# Autodesk Inventor assembly: Lathe Model V3
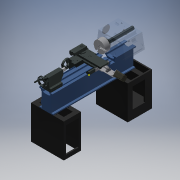
[picture p0: Inventor's stored thumbnail of the model, 180x180]
Saved by Autodesk Inventor 2018 (Build 220112000, 112)
## iProperties
Created: 2017-05-02
Part Number: Lathe Model V3
Document SubType Name: Assembly
Designer: M228544
Author: M228544
## Documents named in this file (28)
- C:\Users\M228299\Documents\GitHub\CNC-Lathe-CAD\CNC Lathe Project\Project Files\Lathe Model 2018.iam
- C:\Users\M228299\Documents\GitHub\CNC-Lathe-CAD\CNC Lathe Project\Project Files\BED.ipt
- C:\Users\M228299\Documents\GitHub\CNC-Lathe-CAD\CNC Lathe Project\Project Files\Bottom-Tool-Bit.ipt
- C:\Users\M228299\Documents\GitHub\CNC-Lathe-CAD\CNC Lathe Project\Project Files\Top-Part-Tool-bit.ipt
- C:\Users\M228299\Documents\GitHub\CNC-Lathe-CAD\CNC Lathe Project\Project Files\tail stock - body part.ipt
- C:\Users\M228299\Documents\GitHub\CNC-Lathe-CAD\CNC Lathe Project\Project Files\Left leg.ipt
- C:\Users\M228299\Documents\GitHub\CNC-Lathe-CAD\CNC Lathe Project\Project Files\Right Leg.ipt
- C:\Users\M228299\Documents\GitHub\CNC-Lathe-CAD\CNC Lathe Project\Project Files\Apron.ipt
- C:\Users\M228299\Documents\GitHub\CNC-Lathe-CAD\CNC Lathe Project\Project Files\Servo Motor\Servo Motor.iam
- C:\Users\M228299\Documents\GitHub\CNC-Lathe-CAD\CNC Lathe Project\Project Files\Ball screw nut and apron join.ipt
- C:\Users\M228299\Documents\GitHub\CNC-Lathe-CAD\CNC Lathe Project\Project Files\barrel.ipt
- C:\Users\M228299\Documents\GitHub\CNC-Lathe-CAD\CNC Lathe Project\Project Files\connecting wheel.ipt
- C:\Users\M228299\Documents\GitHub\CNC-Lathe-CAD\CNC Lathe Project\Project Files\chuck holder.ipt
- C:\Users\M228299\Documents\GitHub\CNC-Lathe-CAD\CNC Lathe Project\Project Files\Chuck shaft.ipt
- C:\Users\M228299\Documents\GitHub\CNC-Lathe-CAD\CNC Lathe Project\Project Files\X axis screw support.ipt
- C:\Users\M228299\Documents\GitHub\CNC-Lathe-CAD\CNC Lathe Project\Project Files\Assembly3.iam
- C:\Users\M228299\Documents\GitHub\CNC-Lathe-CAD\CNC Lathe Project\Project Files\Gearbox Handle.iam
- C:\Users\M228299\Documents\GitHub\CNC-Lathe-CAD\CNC Lathe Project\Project Files\Encoder Mount Hole Plug.ipt
- C:\Users\M228299\Documents\GitHub\CNC-Lathe-CAD\CNC Lathe Project\Project Files\Gearbox.ipt
- C:\Users\M228299\Documents\GitHub\CNC-Lathe-CAD\CNC Lathe Project\Project Files\Encoder Subassembly\Mounting.iam
- C:\Users\M228299\Documents\GitHub\CNC-Lathe-CAD\CNC Lathe Project\Project Files\X-axis Changes\slide-ontop-of-saddle.ipt
- C:\Users\M228299\Documents\GitHub\CNC-Lathe-CAD\CNC Lathe Project\Project Files\X-axis Changes\X Axis Shaft Assembly\short shaft x axis\shaft and nut.iam
- C:\Users\M228299\Documents\GitHub\CNC-Lathe-CAD\CNC Lathe Project\Project Files\X-axis Changes\Ball Screw\Correct nut unmodified ASSembly.iam
- C:\Users\M228299\Documents\GitHub\CNC-Lathe-CAD\CNC Lathe Project\Project Files\X-axis Changes\Ball Screw\X-axis Ball Screw Support.ipt
- C:\Users\M228299\Documents\GitHub\CNC-Lathe-CAD\CNC Lathe Project\Project Files\saddle.ipt
- C:\Users\M228299\Documents\GitHub\CNC-Lathe-CAD\CNC Lathe Project\Project Files\back plate.ipt
- C:\Users\M228299\Documents\GitHub\CNC-Lathe-CAD\CNC Lathe Project\Project Files\front.ipt
- C:\Users\M228299\Documents\GitHub\CNC-Lathe-CAD\CNC Lathe Project\Project Files\polycarbonate cover.ipt
## Components (27 placed, 27 different names)
1. BED:1 — Mate:1, Mate:2, Mate:9, Mate:10, Mate:11, Flush:5, Flush:6, Mate:13, Mate:14, Flush:7, Flush:9
2. saddle:1 — Mate:1, Mate:2, Mate:5, Mate:6, Saddle and Slice on top of saddle, Flush:10, Flush:11, Mate:15, Mate:20, Flush:36, Angle:7, Mate:61, Mate:62
3. Bottom-Tool-Bit:1 — Mate:3, Mate:4, Flush:14
4. Top-Part-Tool-bit:1 — Mate:3, Mate:4, Mate:7, Mate:8, Tool Bit and Slece on top of saddle, Flush:14
5. slide-ontop-of-saddle:1 — Mate:5, Mate:6, Mate:7, Mate:8, Saddle and Slice on top of saddle, Tool Bit and Slece on top of saddle, Mate:70
6. tail stock - body part:1 — Mate:9, Mate:10, Flush:13, Mate:19, Mate:20, Mate:35, Mate:38, Flush:33
7. Gearbox:1 — Mate:11, Flush:5, Flush:13, Mate:19, Mate:21, Mate:39, Mate:40, Rotational:1, Mate:49, Flush:37, Mate:50, Mate:51, Mate:75, Mate:76
8. Left leg:1 — Mate:14, Flush:7, Flush:8, Mate:71, Flush:40
9. Right Leg:1 — Flush:6, Mate:13, Flush:8, Flush:9, Mate:73, Flush:43
10. Apron:1 — Flush:10, Flush:11, Mate:15, Mate:21, Mate:34
11. Ball screw nut and apron join:1 — Mate:34
12. barrel:1 — Mate:35, Mate:36, Mate:37, Rotation/Translation:1, Flush:33
13. connecting wheel:1 — Mate:36, Mate:37, Mate:38, Rotation/Translation:1
14. chuck holder:1 — Mate:39, Mate:40, Mate:41, Mate:42, Mate:48
15. Chuck shaft:1 — Mate:41, Mate:42, Mate:47
16. X axis screw support:1 — Flush:36, Mate:46, Mate:63, Mate:64, Angle:8, Mate:65, Mate:66
17. Servo Motor:2 [sub-assembly] — Mate:46, Angle:7, Mate:65, Mate:66
18. Assembly3:1 [sub-assembly] — Mate:47, Mate:48
19. Gearbox Handle:1 [sub-assembly] — Rotational:1
20. Encoder Mount Hole Plug:1 — Mate:49, Flush:37
21. Mounting:1 [sub-assembly] — Mate:50, Mate:51
22. shaft and nut:1 [sub-assembly] — Mate:61, Mate:62, Mate:63, Mate:64, Mate:67, Mate:69
23. Correct nut unmodified ASSembly:1 [sub-assembly] — Mate:67, Angle:9, Mate:68
24. X-axis Ball Screw Support:1 — Mate:68, Mate:69, Angle:10, Mate:70
25. back plate:1 — Mate:71, Flush:40, Rotational:2, Mate:75
26. front:1 — Mate:73, Flush:43, Mate:76
27. polycarbonate cover:1 — Rotational:2
## Relationships (69: Mate 46, Flush 15, Angle 5, RevoluteJoint 2, RelateRotateTranslate 1)
- Mate:1: BED:1 ↔ saddle:1
- Mate:2: BED:1 ↔ saddle:1
- Mate:3: Bottom-Tool-Bit:1 ↔ Top-Part-Tool-bit:1
- Mate:4: Bottom-Tool-Bit:1 ↔ Top-Part-Tool-bit:1
- Mate:5: saddle:1 ↔ slide-ontop-of-saddle:1
- Mate:6: saddle:1 ↔ slide-ontop-of-saddle:1
- Mate:7: Top-Part-Tool-bit:1 ↔ slide-ontop-of-saddle:1
- Mate:8: Top-Part-Tool-bit:1 ↔ slide-ontop-of-saddle:1
- Mate:9: BED:1 ↔ tail stock - body part:1
- Mate:10: BED:1 ↔ tail stock - body part:1
- Saddle and Slice on top of saddle [Flush]: saddle:1 ↔ slide-ontop-of-saddle:1
- Tool Bit and Slece on top of saddle [Angle] (-90 deg): Top-Part-Tool-bit:1 ↔ slide-ontop-of-saddle:1
- Mate:11 (2 mm): BED:1 ↔ Gearbox:1
- Flush:5: BED:1 ↔ Gearbox:1
- Flush:13 (-22 mm): tail stock - body part:1 ↔ Gearbox:1
- Flush:6: BED:1 ↔ Right Leg:1
- Mate:13: BED:1 ↔ Right Leg:1
- Mate:14: BED:1 ↔ Left leg:1
- Flush:7: BED:1 ↔ Left leg:1
- Flush:8: Left leg:1 ↔ Right Leg:1
- Flush:9 (145 mm): BED:1 ↔ Right Leg:1
- Flush:10: saddle:1 ↔ Apron:1
- Flush:11: saddle:1 ↔ Apron:1
- Mate:15: saddle:1 ↔ Apron:1
- Flush:14: Bottom-Tool-Bit:1 ↔ Top-Part-Tool-bit:1
- Mate:19: tail stock - body part:1 ↔ Gearbox:1
- Mate:20: saddle:1 ↔ tail stock - body part:1
- Mate:21: Gearbox:1 ↔ Apron:1
- Mate:34: Apron:1 ↔ Ball screw nut and apron join:1
- Mate:35: tail stock - body part:1 ↔ barrel:1
- Mate:36: barrel:1 ↔ connecting wheel:1
- Mate:37: barrel:1 ↔ connecting wheel:1
- Mate:38: tail stock - body part:1 ↔ connecting wheel:1
- Rotation/Translation:1 [RelateRotateTranslate] (100 mm): barrel:1 ↔ connecting wheel:1
- Flush:33: tail stock - body part:1 ↔ barrel:1
- Mate:39: Gearbox:1 ↔ chuck holder:1
- Mate:40 (0.46 mm): Gearbox:1 ↔ chuck holder:1
- Mate:41: chuck holder:1 ↔ Chuck shaft:1
- Mate:42 (11.2 mm): chuck holder:1 ↔ Chuck shaft:1
- Flush:36: saddle:1 ↔ X axis screw support:1
- Mate:46: X axis screw support:1 ↔ Servo Motor:2
- Angle:7 (225 deg): saddle:1 ↔ Servo Motor:2
- Mate:47: Chuck shaft:1 ↔ Assembly3:1
- Mate:48: chuck holder:1 ↔ Assembly3:1
- Rotational:1 [RevoluteJoint]: Gearbox:1 ↔ Gearbox Handle:1
- Mate:49: Gearbox:1 ↔ Encoder Mount Hole Plug:1
- Flush:37: Gearbox:1 ↔ Encoder Mount Hole Plug:1
- Mate:50: Gearbox:1 ↔ Mounting:1
- Mate:51: Gearbox:1 ↔ Mounting:1
- Mate:61: saddle:1 ↔ shaft and nut:1
- Mate:62: saddle:1 ↔ shaft and nut:1
- Mate:63: X axis screw support:1 ↔ shaft and nut:1
- Mate:64 (-50 mm): X axis screw support:1 ↔ shaft and nut:1
- Angle:8 (180 deg): X axis screw support:1
- Mate:65: X axis screw support:1 ↔ Servo Motor:2
- Mate:66: X axis screw support:1 ↔ Servo Motor:2
- Mate:67: shaft and nut:1 ↔ Correct nut unmodified ASSembly:1
- Angle:9 (180 deg): Correct nut unmodified ASSembly:1
- Mate:68: Correct nut unmodified ASSembly:1 ↔ X-axis Ball Screw Support:1
- Mate:69: shaft and nut:1 ↔ X-axis Ball Screw Support:1
- Angle:10 (90 deg): X-axis Ball Screw Support:1
- Mate:70 (-261 mm): slide-ontop-of-saddle:1 ↔ X-axis Ball Screw Support:1
- Mate:71: Left leg:1 ↔ back plate:1
- Flush:40: Left leg:1 ↔ back plate:1
- Mate:73: Right Leg:1 ↔ front:1
- Flush:43 (6.4 mm): Right Leg:1 ↔ front:1
- Rotational:2 [RevoluteJoint]: back plate:1 ↔ polycarbonate cover:1
- Mate:75: Gearbox:1 ↔ back plate:1
- Mate:76: Gearbox:1 ↔ front:1
